# Autodesk Inventor assembly: Tornillo Soinfin_v001
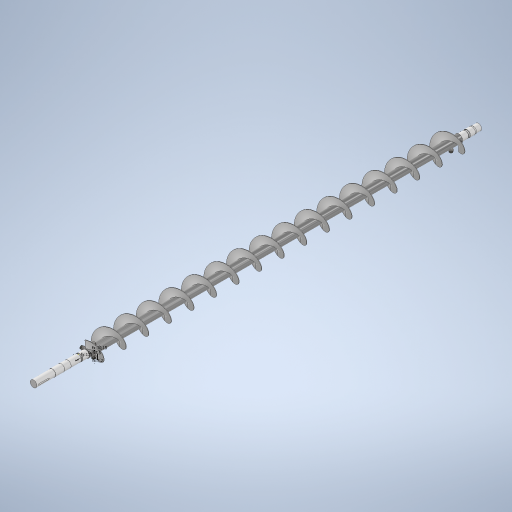
[picture p0: Inventor's stored thumbnail of the model, 512x512]
Saved by Autodesk Inventor 2024 (Build 280153000, 153)
## iProperties
RuleStatus: InUse
Created: 2026-01-08
Part Number: Tornillo Soinfin_v001
Document SubType Name: Assembly
Designer: eduso
Author: eduso
## Documents named in this file (7)
- C:\edusonros_projects\SINFINES_CONRAD\iLogic\Tornillo Sinfin_v001.iam
- C:\edusonros_projects\SINFINES_CONRAD\iLogic\Tubo_Perforado_Base.ipt
- C:\edusonros_projects\SINFINES_CONRAD\iLogic\Mangon_Conducido.ipt
- C:\edusonros_projects\SINFINES_CONRAD\iLogic\Mangon_Conduccion.ipt
- C:\edusonros_projects\SINFINES_CONRAD\iLogic\Espira_01.ipt
- C:\edusonros_projects\SINFINES_CONRAD\iLogic\Espira_01_Parcial.ipt
- C:\edusonros_projects\SINFINES_CONRAD\iLogic\Tornilo+tuerca M12x90.iam
## Components (24 placed, 6 different names)
1. Tubo_Perforado_Base:1 — Mate:1, Mate:2, Mate:3, Mate:4, Mate:5, Mate:6, Tangent:1, Tangent:2, Mate:11, Tangent:3, Mate:12, Tangent:4, Mate:13, Mate:14
2. Mangon_Conducido:1 — Mate:1, Mate:2, Mate:10
3. Mangon_Conduccion:1 — Mate:3, Mate:4, Mate:9
4. Espira_01_Parcial:1 — Mate:13, Mate:14
5. Tornilo+tuerca M12x90:1 [sub-assembly] — Mate:9, Tangent:1
6. Tornilo+tuerca M12x90:2 [sub-assembly] — Mate:12, Tangent:4
7. Tornilo+tuerca M12x90:3 [sub-assembly] — Mate:10, Tangent:2
8. Tornilo+tuerca M12x90:4 [sub-assembly] — Mate:11, Tangent:3
9. Espira_01:1 — Mate:5, Mate:6
10. Espira_01:3
11. Espira_01:4
12. Espira_01:5
13. Espira_01:6
14. Espira_01:7
15. Espira_01:8
16. Espira_01:9
17. Espira_01:10
18. Espira_01:11
19. Espira_01:12
20. Espira_01:13
21. Espira_01:14
22. Espira_01:15
23. Espira_01:16
24. Espira_01:17
## Component patterns: (16 elements, first: Espira_01:1)
## Relationships (16: Mate 12, Tangent 4)
- Mate:1: Tubo_Perforado_Base:1 ↔ Mangon_Conducido:1
- Mate:2: Tubo_Perforado_Base:1 ↔ Mangon_Conducido:1
- Mate:3: Tubo_Perforado_Base:1 ↔ Mangon_Conduccion:1
- Mate:4: Tubo_Perforado_Base:1 ↔ Mangon_Conduccion:1
- Mate:5: Tubo_Perforado_Base:1 ↔ Espira_01:1
- Mate:6: Tubo_Perforado_Base:1 ↔ Espira_01:1
- Mate:9: Mangon_Conduccion:1 ↔ Tornilo+tuerca M12x90:1
- Tangent:1: Tubo_Perforado_Base:1 ↔ Tornilo+tuerca M12x90:1
- Mate:10: Mangon_Conducido:1 ↔ Tornilo+tuerca M12x90:3
- Tangent:2: Tubo_Perforado_Base:1 ↔ Tornilo+tuerca M12x90:3
- Mate:11: Tubo_Perforado_Base:1 ↔ Tornilo+tuerca M12x90:4
- Tangent:3: Tubo_Perforado_Base:1 ↔ Tornilo+tuerca M12x90:4
- Mate:12: Tubo_Perforado_Base:1 ↔ Tornilo+tuerca M12x90:2
- Tangent:4: Tubo_Perforado_Base:1 ↔ Tornilo+tuerca M12x90:2
- Mate:13: Tubo_Perforado_Base:1 ↔ Espira_01_Parcial:1
- Mate:14: Tubo_Perforado_Base:1 ↔ Espira_01_Parcial:1
## Named parameters: Paso_Espira_01 = 175 mm, ø_Ext_Espira_01 = 175 mm, ø_Int_Espira_01 = 60.3 mm, Espesor_Espira_01 = 3.2 mm, Testero_007 = 5 mm, Espacio_008 = 50 mm, Inteerior_Tubo_009 = 80 mm, Cido_Testero_007 = 4 mm, Cido_Espacio_008 = 50 mm, Cido_Inteerior_Tubo_009 = 80 mm, Largo = 2890 mm, DiametroExterior = 60.3 mm, Espesor = 3.2 mm, DiametroInterior = 53.9 mm, Num_Espiras = 16, Resto = 90 mm
